# Autodesk Inventor assembly: palma-motores
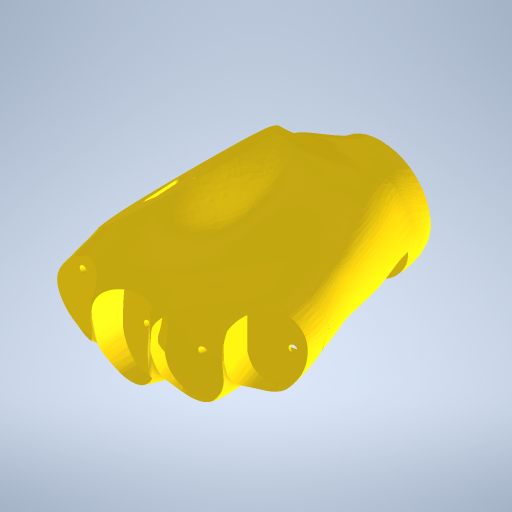
[picture p0: Inventor's stored thumbnail of the model, 512x512]
Saved by Autodesk Inventor 2024 (Build 280153000, 153)
## iProperties
Created: 2023-04-25
Part Number: palma-motores
Document SubType Name: Assembly
Designer: david
Author: david
## Documents named in this file (3)
- X:\palma-motores.iam
- X:\Palm\Righ_Hand_Palm.ipt
- X:\Motor-case-v2.iam
## Components (6 placed, 2 different names)
1. Righ_Hand_Palm:1 — Mate:1, Mate:2, Mate:3, Mate:4, Mate:5
2. Motor-case-v2:4 [sub-assembly] — Mate:3
3. Motor-case-v2:6 [sub-assembly] — Mate:2
4. Motor-case-v2:7 [sub-assembly] — Mate:4
5. Motor-case-v2:8 [sub-assembly] — Mate:5
6. Motor-case-v2:9 [sub-assembly] — Mate:1
## Relationships (5: Mate 5)
- Mate:1: Righ_Hand_Palm:1 ↔ Motor-case-v2:9
- Mate:2: Righ_Hand_Palm:1 ↔ Motor-case-v2:6
- Mate:3: Righ_Hand_Palm:1 ↔ Motor-case-v2:4
- Mate:4: Righ_Hand_Palm:1 ↔ Motor-case-v2:7
- Mate:5: Righ_Hand_Palm:1 ↔ Motor-case-v2:8
